# Autodesk Inventor assembly: Pirani Gauge
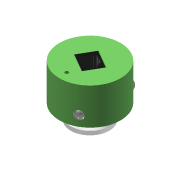
[picture p0: Inventor's stored thumbnail of the model, 180x180]
Saved by Autodesk Inventor 2020 (Build 240168000, 168)
## iProperties
Created: 2018-03-06
Part Number: Pirani Gauge
Document SubType Name: Assembly
Designer: Alex
Author: Alex
## Documents named in this file (11)
- C:\Users\amsmi\Google Drive\Pirani Gauge\Pirani Gauge Modeling\Gauge Rev 3\Pirani Gauge.iam
- C:\Users\amsmi\Google Drive\Pirani Gauge\Pirani Gauge Modeling\Gauge Rev 3\#22 o-ring.ipt
- C:\Users\amsmi\Google Drive\Pirani Gauge\Pirani Gauge Modeling\Gauge Rev 3\Filament Board.iam
- C:\Users\amsmi\Google Drive\Pirani Gauge\Pirani Gauge Modeling\Gauge Rev 3\RJ12 - Straight.ipt
- C:\Users\amsmi\Google Drive\Pirani Gauge\Pirani Gauge Modeling\Gauge Rev 3\Board Spacer - 2.ipt
- C:\Users\amsmi\Google Drive\Pirani Gauge\Pirani Gauge Modeling\Gauge Rev 3\Housing - 3,2.ipt
- C:\Users\amsmi\Google Drive\Pirani Gauge\Pirani Gauge Modeling\Gauge Rev 3\Power Supply Board.iam
- C:\Users\amsmi\Google Drive\Pirani Gauge\Pirani Gauge Modeling\Gauge Rev 3\2-56 1-2in length PHS.ipt
- C:\Users\amsmi\Google Drive\Pirani Gauge\Pirani Gauge Modeling\Gauge Rev 3\4-40 1-4in length PHS.ipt
- C:\Users\amsmi\Google Drive\Pirani Gauge\Pirani Gauge Modeling\Gauge Rev 3\Vacuum Housing - KF.ipt
- C:\Users\amsmi\Google Drive\Pirani Gauge\Pirani Gauge Modeling\Gauge Rev 3\Filament - updated.ipt
## Components (14 placed, 10 different names)
1. Vacuum Housing - KF:1 — Mate:41, Mate:42, Mate:43, Mate:44, Tangent:5, Mate:45, Mate:46, Mate:47
2. #22 o-ring:1 — Mate:44, Tangent:5
3. Filament Board:1 [sub-assembly] — Mate:8, Mate:9, Mate:10, Mate:18, Mate:20, Mate:23, Mate:47
4. Filament - updated:1 — Mate:8, Mate:9, Mate:10
5. RJ12 - Straight:1 — Mate:28, Mate:29, Angle:1
6. Board Spacer - 2:1 — Mate:18, Mate:20, Mate:23, Mate:24, Mate:25, Mate:26, Mate:27, Mate:39, Mate:40
7. Housing - 3,2:1 — Mate:24, Mate:36, Mate:37, Mate:38, Mate:39, Mate:40, Tangent:2, Tangent:3, Tangent:4
8. Power Supply Board:1 [sub-assembly] — Mate:25, Mate:26, Mate:27, Mate:28, Mate:29, Angle:1, Mate:30, Mate:31, Mate:32, Mate:33, Mate:34, Mate:35
9. 2-56 1-2in length PHS:1 — Mate:30, Mate:33, Mate:45
10. 2-56 1-2in length PHS:2 — Mate:31, Mate:34
11. 2-56 1-2in length PHS:3 — Mate:32, Mate:35, Mate:46
12. 4-40 1-4in length PHS:1 — Mate:38, Tangent:3
13. 4-40 1-4in length PHS:2 — Mate:37, Tangent:4
14. 4-40 1-4in length PHS:3 — Mate:36, Tangent:2
## Relationships (35: Mate 30, Tangent 4, Angle 1)
- Mate:8: Filament Board:1 ↔ Filament - updated:1
- Mate:9: Filament Board:1 ↔ Filament - updated:1
- Mate:10 (0.508 mm): Filament Board:1 ↔ Filament - updated:1
- Mate:18: Filament Board:1 ↔ Board Spacer - 2:1
- Mate:20: Filament Board:1 ↔ Board Spacer - 2:1
- Mate:23: Filament Board:1 ↔ Board Spacer - 2:1
- Mate:24: Board Spacer - 2:1 ↔ Housing - 3,2:1
- Mate:25: Board Spacer - 2:1 ↔ Power Supply Board:1
- Mate:26: Board Spacer - 2:1 ↔ Power Supply Board:1
- Mate:27: Board Spacer - 2:1 ↔ Power Supply Board:1
- Mate:28: RJ12 - Straight:1 ↔ Power Supply Board:1
- Mate:29: RJ12 - Straight:1 ↔ Power Supply Board:1
- Angle:1 (0 deg): RJ12 - Straight:1 ↔ Power Supply Board:1
- Mate:30: Power Supply Board:1 ↔ 2-56 1-2in length PHS:1
- Mate:31: Power Supply Board:1 ↔ 2-56 1-2in length PHS:2
- Mate:32: Power Supply Board:1 ↔ 2-56 1-2in length PHS:3
- Mate:33: Power Supply Board:1 ↔ 2-56 1-2in length PHS:1
- Mate:34: Power Supply Board:1 ↔ 2-56 1-2in length PHS:2
- Mate:35: Power Supply Board:1 ↔ 2-56 1-2in length PHS:3
- Mate:36: Housing - 3,2:1 ↔ 4-40 1-4in length PHS:3
- Mate:37: Housing - 3,2:1 ↔ 4-40 1-4in length PHS:2
- Mate:38: Housing - 3,2:1 ↔ 4-40 1-4in length PHS:1
- Mate:39: Board Spacer - 2:1 ↔ Housing - 3,2:1
- Mate:40: Board Spacer - 2:1 ↔ Housing - 3,2:1
- Tangent:2: Housing - 3,2:1 ↔ 4-40 1-4in length PHS:3
- Tangent:3: Housing - 3,2:1 ↔ 4-40 1-4in length PHS:1
- Tangent:4: Housing - 3,2:1 ↔ 4-40 1-4in length PHS:2
- Mate:41: Vacuum Housing - KF:1
- Mate:42: Vacuum Housing - KF:1
- Mate:43: Vacuum Housing - KF:1
- Mate:44: Vacuum Housing - KF:1 ↔ #22 o-ring:1
- Tangent:5: Vacuum Housing - KF:1 ↔ #22 o-ring:1
- Mate:45: Vacuum Housing - KF:1 ↔ 2-56 1-2in length PHS:1
- Mate:46: Vacuum Housing - KF:1 ↔ 2-56 1-2in length PHS:3
- Mate:47: Vacuum Housing - KF:1 ↔ Filament Board:1
